# Autodesk Inventor assembly: Cabin Assembly
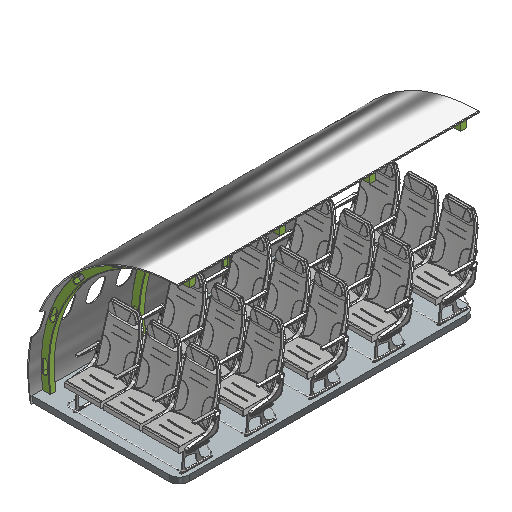
[picture p0: Inventor's stored thumbnail of the model, 512x512]
Saved by Autodesk Inventor 2026.2 (Build 302298000, 298)
## iProperties
Created: 2026-01-10
Part Number: Cabin Assembly
Document SubType Name: Assembly
Designer: andyeske
Author: andyeske
## Documents named in this file (3)
- C:\Users\andyeske\Inventor\Cabin Assembly.iam
- C:\Users\andyeske\Inventor\Fuselage.ipt
- C:\Users\andyeske\Inventor\Economy Seat.ipt
## Components (2 placed, 2 different names)
1. Fuselage:1 — Mate:1, Flush:1
2. Economy Seat:1 — Mate:1, Flush:1
## Relationships (2: Mate 1, Flush 1)
- Mate:1: Fuselage:1 ↔ Economy Seat:1
- Flush:1 (50.8 mm): Fuselage:1 ↔ Economy Seat:1
